# Autodesk Inventor assembly: Hinge assembly
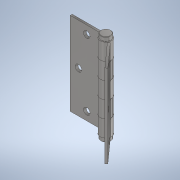
[picture p0: Inventor's stored thumbnail of the model, 180x180]
Saved by Autodesk Inventor 2021 (Build 250183000, 183)
## iProperties
Created: 2021-07-31
Part Number: Hinge assembly
Document SubType Name: Assembly
Designer: Shammy Haider
Author: Shammy Haider
## Documents named in this file (4)
- D:\Designing\Autodesk inventor\Wood Door\Hinge assembly.iam
- D:\Designing\Autodesk inventor\Wood Door\Connecting rod hinge.ipt
- D:\Designing\Autodesk inventor\Wood Door\Hinge1.ipt
- D:\Designing\Autodesk inventor\Wood Door\Hinge2.ipt
## Components (3 placed, 3 different names)
1. Connecting rod hinge:1 — Mate:3, Mate:4
2. Hinge1:1 — Mate:1, Mate:2, Mate:3, Mate:4
3. Hinge2:1 — Mate:1, Mate:2
## Relationships (4: Mate 4)
- Mate:1: Hinge1:1 ↔ Hinge2:1
- Mate:2: Hinge1:1 ↔ Hinge2:1
- Mate:3: Connecting rod hinge:1 ↔ Hinge1:1
- Mate:4: Connecting rod hinge:1 ↔ Hinge1:1
